# Autodesk Inventor assembly: ajuste aguejero eje
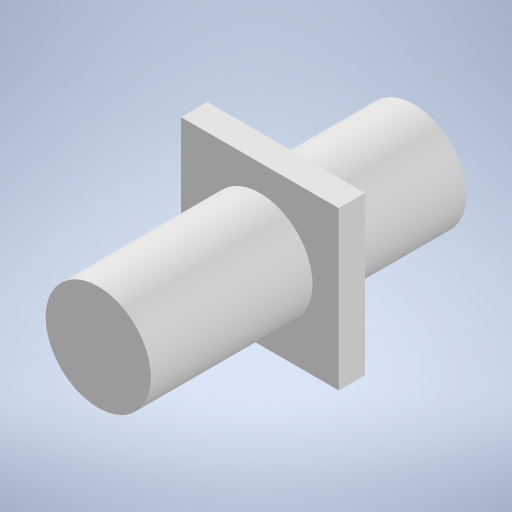
[picture p0: Inventor's stored thumbnail of the model, 512x512]
Saved by Autodesk Inventor 2023.2 (Build 272271030, 271C)
## iProperties
Created: 2023-10-02
Part Number: ajuste aguejero eje
Document SubType Name: Assembly
Designer: Cris Pat
Author: Cris Pat
## Documents named in this file (3)
- C:\Users\Cris Pat\Desktop\U\Semestre_10\Disenio_y_manufactura\despues_descanso_eje\ajuste aguejero eje.iam
- C:\Users\Cris Pat\Desktop\U\Semestre_10\Disenio_y_manufactura\despues_descanso_eje\AGUJERO.ipt
- C:\Users\Cris Pat\Desktop\U\Semestre_10\Disenio_y_manufactura\despues_descanso_eje\eje_Agujero.ipt
## Components (2 placed, 2 different names)
1. AGUJERO:1 — Flush:1, Mate:1
2. eje_Agujero:1 — Flush:1, Mate:1
## Relationships (2: Flush 1, Mate 1)
- Flush:1: AGUJERO:1 ↔ eje_Agujero:1
- Mate:1: AGUJERO:1 ↔ eje_Agujero:1
